# Autodesk Inventor assembly: 조립품1
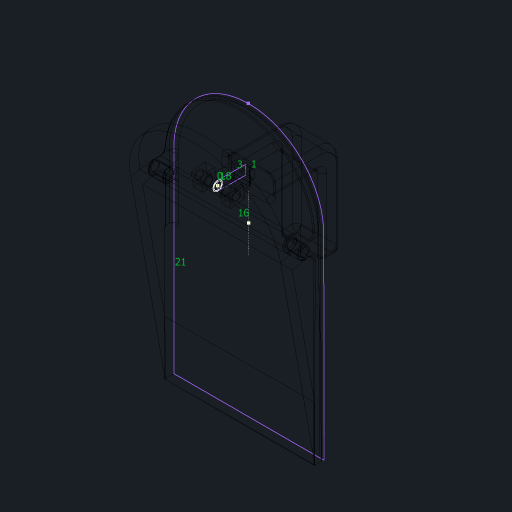
[picture p0: Inventor's stored thumbnail of the model, 512x512]
Saved by Autodesk Inventor 2024.1 (Build 281209000, 209)
## iProperties
Created: 2024-01-27
Part Number: 조립품1
Document SubType Name: Assembly
Designer: likek
Author: likek
## Documents named in this file (4)
- C:\Users\likek\Videos\Modeling\IKEA 페그보드 시제품\조립품1.iam
- C:\Users\likek\Videos\Modeling\IKEA 페그보드 시제품\집게 베이스.ipt
- C:\Users\likek\Videos\Modeling\IKEA 페그보드 시제품\집게 이동.ipt
- C:\Users\likek\Videos\Modeling\IKEA 페그보드 시제품\집게 고정.ipt
## Components (3 placed, 3 different names)
1. 집게 베이스:1 — 삽입:1, 각도:1
2. 집게 이동:1 — 삽입:1, 삽입:2, 각도:1
3. 집게 고정:1 — 삽입:2
## Relationships (3: Insert 2, Angle 1)
- 삽입:1 [Insert]: 집게 베이스:1 ↔ 집게 이동:1
- 삽입:2 [Insert]: 집게 이동:1 ↔ 집게 고정:1
- 각도:1 [Angle] (180.2558 deg): 집게 베이스:1 ↔ 집게 이동:1
